# Autodesk Inventor assembly: LRT
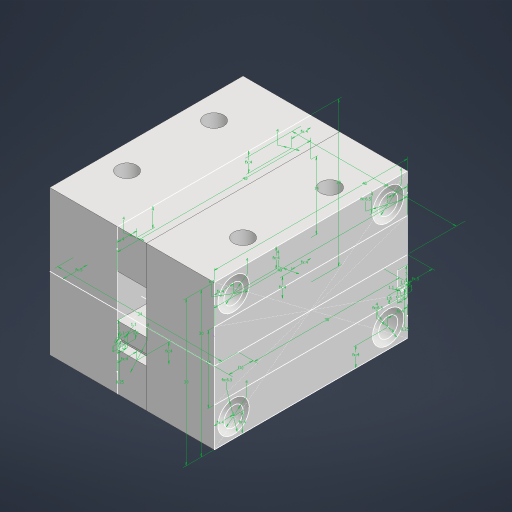
[picture p0: Inventor's stored thumbnail of the model, 512x512]
Saved by Autodesk Inventor 2024.2 (Build 282272000, 272)
## iProperties
Created: 2024-09-29
Part Number: LRT
Document SubType Name: Assembly
Designer: jerem
Author: jerem
## Documents named in this file (3)
- C:\Users\jerem\Desktop\LRT.iam
- C:\Users\jerem\Desktop\LRT_Back.ipt
- C:\Users\jerem\Desktop\LRT_Face.ipt
## Components (2 placed, 2 different names)
1. LRT_Back:1 — Mate:2, Mate:3, Mate:4
2. LRT_Face:1 — Mate:2, Mate:3, Mate:4
## Relationships (3: Mate 3)
- Mate:2: LRT_Back:1 ↔ LRT_Face:1
- Mate:3: LRT_Back:1 ↔ LRT_Face:1
- Mate:4: LRT_Back:1 ↔ LRT_Face:1
